# Autodesk Inventor assembly: Design-Project-EJT
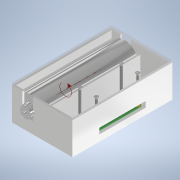
[picture p0: Inventor's stored thumbnail of the model, 180x180]
Saved by Autodesk Inventor 2022 (Build 260153000, 153)
## iProperties
Company: El Camino College
Created: 2022-12-17
Part Number: Design-Project-EJT
Document SubType Name: Assembly
Designer: Edgar Tejada
Project: Parametric-Modeling
Author: Edgar Tejada
Title: Battery-Pack
## Documents named in this file (6)
- G:\Documents\Inventor HW\Parametric-Modeling\BatteryPack\Design-Project-EJT.iam
- G:\Documents\Inventor HW\Parametric-Modeling\BatteryPack\Battery-Pack-Bottom-Shell.ipt
- G:\Documents\Inventor HW\Parametric-Modeling\BatteryPack\Battery-Pack-38120s-10Ah.ipt
- G:\Documents\Inventor HW\Parametric-Modeling\BatteryPack\Raspberry_Pi_Zero_Board.ipt
- G:\Documents\Inventor HW\Parametric-Modeling\BatteryPack\Battery-Pack-Top-Lid.ipt
- C:\Users\brev\Documents\Inventor\Content Center Files\R2022\en-US\AS 1427(03)\AS 1427 - M3 x 50(1).ipt
## Components (8 placed, 5 different names)
1. Battery Pack Bottom-Shell:2 — Mate:1, Cylindrical:1, Mate:2, Mate:3, Mate:4, Mate:5, Mate:6, Mate:7
2. Battery-Pack-38120s-10Ah:1 — Mate:1, Cylindrical:1
3. Raspberry_Pi_Zero_Board:1 — Mate:2, Mate:3, Mate:4
4. Battery-Pack-Top-Lid:1 — Mate:5, Rigid:1, Rigid:2, Rigid:3, Rigid:4
5. AS 1427 - Metric M3 x 50:1 — Rigid:4
6. AS 1427 - Metric M3 x 50:2 — Rigid:3
7. AS 1427 - Metric M3 x 50:3 — Rigid:2, Mate:7
8. AS 1427 - Metric M3 x 50:4 — Rigid:1, Mate:6
## Relationships (12: Mate 7, WeldJoint 4, CylindricalJoint 1)
- Mate:1: Battery Pack Bottom-Shell:2 ↔ Battery-Pack-38120s-10Ah:1
- Cylindrical:1: Battery Pack Bottom-Shell:2 ↔ Battery-Pack-38120s-10Ah:1
- Mate:2: Battery Pack Bottom-Shell:2 ↔ Raspberry_Pi_Zero_Board:1
- Mate:3: Battery Pack Bottom-Shell:2 ↔ Raspberry_Pi_Zero_Board:1
- Mate:4: Battery Pack Bottom-Shell:2 ↔ Raspberry_Pi_Zero_Board:1
- Mate:5: Battery Pack Bottom-Shell:2 ↔ Battery-Pack-Top-Lid:1
- Rigid:1 [WeldJoint] (1 mm): Battery-Pack-Top-Lid:1 ↔ AS 1427 - Metric M3 x 50:4
- Rigid:2 [WeldJoint] (1 mm): Battery-Pack-Top-Lid:1 ↔ AS 1427 - Metric M3 x 50:3
- Rigid:3 [WeldJoint] (1 mm): Battery-Pack-Top-Lid:1 ↔ AS 1427 - Metric M3 x 50:2
- Rigid:4 [WeldJoint] (1 mm): Battery-Pack-Top-Lid:1 ↔ AS 1427 - Metric M3 x 50:1
- Mate:6: Battery Pack Bottom-Shell:2 ↔ AS 1427 - Metric M3 x 50:4
- Mate:7: Battery Pack Bottom-Shell:2 ↔ AS 1427 - Metric M3 x 50:3
